# Autodesk Inventor assembly: Plane_body_pattern
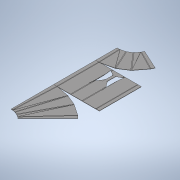
[picture p0: Inventor's stored thumbnail of the model, 180x180]
Saved by Autodesk Inventor 2020 (Build 240168000, 168)
## iProperties
Created: 2020-03-03
Part Number: Plane_body_pattern
Document SubType Name: Assembly
Designer: valem
Author: valem
## Documents named in this file (4)
- D:\Planes\Cardboard_glider_1\Plane_body_pattern.iam
- D:\Planes\Cardboard_glider_1\cabin_unwrap.ipt
- D:\Planes\Cardboard_glider_1\main_body_unwrap.ipt
- D:\Planes\Cardboard_glider_1\tail_unwrap.ipt
## Components (3 placed, 3 different names)
1. Cabin_unwrap:1 — Mate:1, Mate:4, Mate:5
2. Main_body_unwrap:1 — Mate:2, Mate:4, Mate:5, Mate:6, Mate:7
3. Tail_unwrap:1 — Mate:3, Mate:6, Mate:7
## Relationships (7: Mate 7)
- Mate:1: Cabin_unwrap:1
- Mate:2: Main_body_unwrap:1
- Mate:3: Tail_unwrap:1
- Mate:4: Cabin_unwrap:1 ↔ Main_body_unwrap:1
- Mate:5: Cabin_unwrap:1 ↔ Main_body_unwrap:1
- Mate:6: Main_body_unwrap:1 ↔ Tail_unwrap:1
- Mate:7: Main_body_unwrap:1 ↔ Tail_unwrap:1
